# Autodesk Inventor assembly: Carrier Assembly
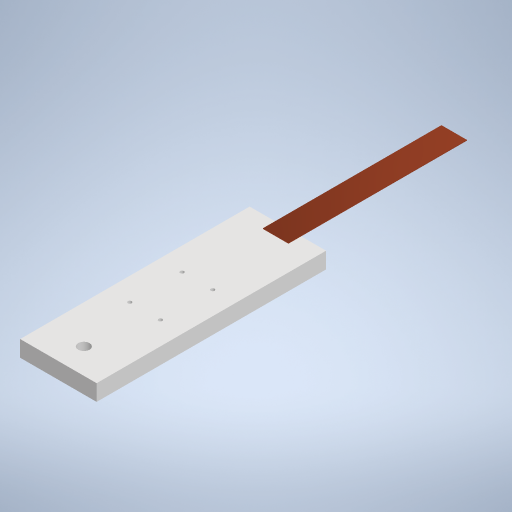
[picture p0: Inventor's stored thumbnail of the model, 512x512]
Saved by Autodesk Inventor 2023 (Build 270158000, 158)
## iProperties
Created: 2023-03-15
Part Number: Carrier Assembly
Document SubType Name: Assembly
Designer: Caleb
Author: Caleb
## Documents named in this file (3)
- C:\Users\Caleb\Desktop\nebraska-silicon-lab\Hardware\TFPX\Carrier Wirebonding Plate\Carrier Assembly.iam
- C:\Users\Caleb\Desktop\nebraska-silicon-lab\Hardware\TFPX\Carrier Wirebonding Plate\Carrier.ipt
- C:\Users\Caleb\Desktop\nebraska-silicon-lab\Hardware\TFPX\Carrier Wirebonding Plate\Pigtail.ipt
## Components (2 placed, 2 different names)
1. Carrier:1 — Mate:1, Mate:2
2. Pigtail:1 — Mate:1, Mate:2
## Relationships (2: Mate 2)
- Mate:1: Carrier:1 ↔ Pigtail:1
- Mate:2 (-5 mm): Carrier:1 ↔ Pigtail:1
